# Autodesk Inventor assembly: Assembly2
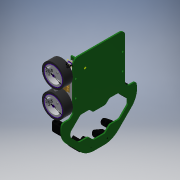
[picture p0: Inventor's stored thumbnail of the model, 180x180]
Saved by Autodesk Inventor 2016 (Build 200138000, 138)
## iProperties
Created: 2017-05-26
Part Number: Assembly2
Material: Ogólny
Document SubType Name: Assembly
Designer: Karol
Author: Karol
## Documents named in this file (17)
- D:\Git\MicromouseDixi\hardware\models\Dixi.iam
- D:\Git\MicromouseDixi\hardware\models\wheel.ipt
- D:\Git\MicromouseDixi\hardware\models\togh.ipt
- D:\Git\MicromouseDixi\hardware\models\bolt.ipt
- D:\Git\MicromouseDixi\hardware\models\magnet.ipt
- D:\Git\MicromouseDixi\hardware\models\mainpcb.ipt
- D:\Git\MicromouseDixi\hardware\models\motor.ipt
- D:\Git\MicromouseDixi\hardware\models\top_mount.ipt
- D:\Git\MicromouseDixi\hardware\models\XSM_0203_03_1.ipt
- D:\Git\MicromouseDixi\hardware\models\XFM_020406_03_233.ipt
- D:\Git\MicromouseDixi\hardware\models\enc_pcb.ipt
- D:\Git\MicromouseDixi\hardware\models\tyre.ipt
- D:\Git\MicromouseDixi\hardware\models\Dixi\Design Accelerator\Spur Gears4.iam
- D:\Git\MicromouseDixi\hardware\models\Dixi\Design Accelerator\Spur Gears3.iam
- D:\Git\MicromouseDixi\hardware\models\magnet_holder.ipt
- D:\Git\MicromouseDixi\hardware\models\tssop14.iam
- D:\Git\MicromouseDixi\hardware\models\led_mount.ipt
## Components (27 placed, 15 different names)
1. mainpcb:1 — Rotational:1, Rigid:47, Mate:1, Mate:2, Rigid:54
2. bolt:3 — Rigid:15, Rigid:45, Rotational:2
3. bolt:4 — Rigid:14, Rigid:46, Rigid:51, Rigid:52
4. wheel:3 — Rigid:15, Rigid:50
5. wheel:4 — Rigid:14, Rigid:49
6. magnet:4 — Rigid:53
7. togh:2 — Rigid:39, Rigid:40, Rigid:41, Rigid:44, Rotational:1, Rigid:47
8. motor:1 — Rigid:39, Rotational:3
9. top_mount:1 — Rigid:40
10. XSM_0203_03_1:1 — Rigid:42, Rigid:45
11. XFM_020406_03_233:1 — Rigid:41, Rigid:42
12. XSM_0203_03_1:2 — Rigid:46
13. XFM_020406_03_233:2 — Rigid:44
14. enc_pcb:1 — Planar:1, Rigid:54
15. tyre:1 — Rigid:49
16. tyre:2 — Rigid:50
17. Spur Gears:2 [sub-assembly] — Rigid:51
18. Spur Gears:7 [sub-assembly] — Rotational:2
19. Spur Gears:8 [sub-assembly] — Rotational:3
20. magnet_holder:1 — Rigid:52, Rigid:53
21. tssop14:1 [sub-assembly] — Planar:1
22. led_mount:1
23. led_mount:2
24. led_mount:3
25. led_mount:4
26. led_mount:5
27. led_mount:6
## Relationships (23: WeldJoint 17, RevoluteJoint 3, Mate 2, PlanarJoint 1)
- Rigid:14 [WeldJoint] (-1.8 mm): bolt:4 ↔ wheel:4
- Rigid:15 [WeldJoint] (-1.8 mm): bolt:3 ↔ wheel:3
- Rigid:39 [WeldJoint]: togh:2 ↔ motor:1
- Rigid:40 [WeldJoint]: togh:2 ↔ top_mount:1
- Rigid:41 [WeldJoint]: togh:2 ↔ XFM_020406_03_233:1
- Rigid:42 [WeldJoint] (-1.5 mm): XSM_0203_03_1:1 ↔ XFM_020406_03_233:1
- [WeldJoint]: XSM_0203_03_1:2 ↔ XFM_020406_03_233:2
- Rigid:44 [WeldJoint] (1 mm): togh:2 ↔ XFM_020406_03_233:2
- Rigid:45 [WeldJoint] (1.5 mm): bolt:3 ↔ XSM_0203_03_1:1
- Rigid:46 [WeldJoint]: bolt:4 ↔ XSM_0203_03_1:2
- Rotational:1 [RevoluteJoint]: mainpcb:1 ↔ togh:2
- Rigid:47 [WeldJoint]: mainpcb:1 ↔ togh:2
- Rigid:49 [WeldJoint]: wheel:4 ↔ tyre:1
- Rigid:50 [WeldJoint]: wheel:3 ↔ tyre:2
- Mate:1: mainpcb:1
- Mate:2: mainpcb:1
- Rotational:2 [RevoluteJoint] (1.5 mm): bolt:3 ↔ Spur Gears:7
- Rigid:51 [WeldJoint] (1.5 mm): bolt:4 ↔ Spur Gears:2
- Rotational:3 [RevoluteJoint] (-3.7 mm): motor:1 ↔ Spur Gears:8
- Rigid:52 [WeldJoint]: bolt:4 ↔ magnet_holder:1
- Rigid:53 [WeldJoint]: magnet:4 ↔ magnet_holder:1
- Planar:1: enc_pcb:1 ↔ tssop14:1
- Rigid:54 [WeldJoint]: mainpcb:1 ↔ enc_pcb:1
## Named parameters: d111_d4 = -1.8 mm, d112_d5 = 0.127925 deg, d113_d6 = -1.8 mm, d114_d7 = -6.839272 deg, d234_d233 = 0 mm
